# Autodesk Inventor assembly: 0_95x_iris_macro_detection_path
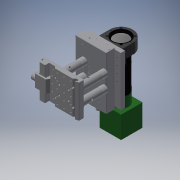
[picture p0: Inventor's stored thumbnail of the model, 180x180]
Saved by Autodesk Inventor 2019 (Build 230136000, 136)
## iProperties
Created: 2019-09-24
Part Number: 0_95x_iris_macro_detection_path
Document SubType Name: Assembly
Designer: voigt
Author: voigt
## Documents named in this file (9)
- J:\Microscope_Design\CAD_Files\mesoSPIM_design_V5.2\mesoSPIM\detection_path\macro_detection_path\0_95x_iris_macro_detection_path.iam
- J:\Microscope_Design\CAD_Files\mesoSPIM_design_V5.2\library\Edmund_Optics\telecentric_objectives\62902_0_9x_F-Mount_PlatinumTL_Telecentric_lens.ipt
- J:\Microscope_Design\CAD_Files\mesoSPIM_design_V5.2\library\Edmund_Optics\telecentric_objectives\56025_mounting_clamp_65mm_diameter.ipt
- J:\Microscope_Design\CAD_Files\mesoSPIM_design_V5.2\mesoSPIM\detection_path\macro_detection_path\MacroBasePlate_V1.ipt
- J:\Microscope_Design\CAD_Files\mesoSPIM_design_V5.2\library\Physik_Instrumente\M-605.2DD-simplified.ipt
- J:\Microscope_Design\CAD_Files\mesoSPIM_design_V5.2\library\Thorlabs\posts\1_inch_posts\RS3P_M.ipt
- J:\Microscope_Design\CAD_Files\mesoSPIM_design_V5.2\library\Newport\X95_carriers\newport_M-CXL95-120.ipt
- J:\Microscope_Design\CAD_Files\mesoSPIM_design_V5.2\library\Photometrics\Iris15_Volume_Incorrect.ipt
- J:\Microscope_Design\CAD_Files\mesoSPIM_design_V5.2\library\Thorlabs\posts\1_inch_post_spacers\RS10M.ipt
## Components (18 placed, 8 different names)
1. 62902_0_9x_F-Mount_PlatinumTL_Telecentric_lens:1 — Mate:1, Mate:2, Flush:2, Mate:20, Mate:21
2. 56025_mounting_clamp_65mm_diameter:1 — Mate:1, Angle:1, Flush:2, Mate:4, Flush:4
3. MacroBasePlate_V1:1 — Mate:4, Flush:3, Flush:4, Mate:5, Mate:8
4. M-605.2DD-simplified:1 — Mate:5, Mate:6, Mate:7, Mate:8, Mate:9, Mate:10, Mate:11, Mate:12, Mate:13, Mate:14, Mate:15, Mate:16
5. RS3P_M:1 — Mate:9, Mate:10, Mate:19, Mate:24, Mate:25
6. RS3P_M:2 — Mate:11, Mate:12, Mate:36, Mate:37
7. RS3P_M:3 — Mate:15, Mate:16, Mate:17, Mate:28, Mate:29
8. RS3P_M:4 — Mate:13, Mate:14, Mate:32, Mate:33
9. newport_M-CXL95-120:1 — Mate:17, Angle:2, Mate:18, Mate:19
10. Iris15_Volume_Incorrect:1 — Mate:20, Mate:21
11. RS10M:1 — Mate:22, Mate:23, Mate:24, Mate:25
12. RS10M:2 — Mate:22, Mate:23
13. RS10M:3 — Mate:28, Mate:29
14. RS10M:4
15. RS10M:5 — Mate:32, Mate:33
16. RS10M:6
17. RS10M:7 — Mate:36, Mate:37
18. RS10M:8
## Relationships (44: Mate 37, Flush 5, Angle 2)
- Mate:1: 62902_0_9x_F-Mount_PlatinumTL_Telecentric_lens:1 ↔ 56025_mounting_clamp_65mm_diameter:1
- Flush:1
- Angle:1 (0 deg): 56025_mounting_clamp_65mm_diameter:1
- Mate:2: 62902_0_9x_F-Mount_PlatinumTL_Telecentric_lens:1
- Mate:3
- Flush:2: 62902_0_9x_F-Mount_PlatinumTL_Telecentric_lens:1 ↔ 56025_mounting_clamp_65mm_diameter:1
- Mate:4: 56025_mounting_clamp_65mm_diameter:1 ↔ MacroBasePlate_V1:1
- Flush:3 (-62.5 mm): MacroBasePlate_V1:1
- Flush:4 (-10 mm): 56025_mounting_clamp_65mm_diameter:1 ↔ MacroBasePlate_V1:1
- Flush:5
- Mate:5: MacroBasePlate_V1:1 ↔ M-605.2DD-simplified:1
- Mate:6: M-605.2DD-simplified:1
- Mate:7: M-605.2DD-simplified:1
- Mate:8: MacroBasePlate_V1:1 ↔ M-605.2DD-simplified:1
- Mate:9 (20 mm): M-605.2DD-simplified:1 ↔ RS3P_M:1
- Mate:10: M-605.2DD-simplified:1 ↔ RS3P_M:1
- Mate:11 (20 mm): M-605.2DD-simplified:1 ↔ RS3P_M:2
- Mate:12: M-605.2DD-simplified:1 ↔ RS3P_M:2
- Mate:13 (20 mm): M-605.2DD-simplified:1 ↔ RS3P_M:4
- Mate:14: M-605.2DD-simplified:1 ↔ RS3P_M:4
- Mate:15 (20 mm): M-605.2DD-simplified:1 ↔ RS3P_M:3
- Mate:16: M-605.2DD-simplified:1 ↔ RS3P_M:3
- Mate:17: RS3P_M:3 ↔ newport_M-CXL95-120:1
- Angle:2 (0 deg): newport_M-CXL95-120:1
- Mate:18: newport_M-CXL95-120:1
- Mate:19 (-35 mm): RS3P_M:1 ↔ newport_M-CXL95-120:1
- Mate:20: 62902_0_9x_F-Mount_PlatinumTL_Telecentric_lens:1 ↔ Iris15_Volume_Incorrect:1
- Mate:21: 62902_0_9x_F-Mount_PlatinumTL_Telecentric_lens:1 ↔ Iris15_Volume_Incorrect:1
- Mate:22: RS10M:1 ↔ RS10M:2
- Mate:23: RS10M:1 ↔ RS10M:2
- Mate:24: RS3P_M:1 ↔ RS10M:1
- Mate:25: RS3P_M:1 ↔ RS10M:1
- [Mate]: RS10M:3 ↔ RS10M:4
- [Mate]: RS10M:3 ↔ RS10M:4
- Mate:28: RS3P_M:3 ↔ RS10M:3
- Mate:29: RS3P_M:3 ↔ RS10M:3
- [Mate]: RS10M:5 ↔ RS10M:6
- [Mate]: RS10M:5 ↔ RS10M:6
- Mate:32: RS3P_M:4 ↔ RS10M:5
- Mate:33: RS3P_M:4 ↔ RS10M:5
- [Mate]: RS10M:7 ↔ RS10M:8
- [Mate]: RS10M:7 ↔ RS10M:8
- Mate:36: RS3P_M:2 ↔ RS10M:7
- Mate:37: RS3P_M:2 ↔ RS10M:7
## Named parameters: d32_d29 = 0 mm, d33_d28 = 0 mm, d36_d32_d29 = 0 mm, d37_d33_d28 = 0 mm, d40_d36_d32_d29 = 0 mm, d41_d37_d33_d28 = 0 mm
